# Autodesk Inventor assembly: Assembly
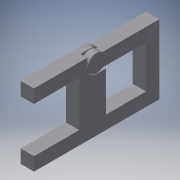
[picture p0: Inventor's stored thumbnail of the model, 180x180]
Saved by Autodesk Inventor 2019 (Build 230136000, 136)
## iProperties
Created: 2018-08-02
Part Number: Assembly
Document SubType Name: Assembly
Designer: zacha
Author: zacha
## Documents named in this file (3)
- F:\SkyDrive\Projects\Cable Guides\Home desk\Assembly.iam
- F:\SkyDrive\Projects\Cable Guides\Home desk\Main.ipt
- F:\SkyDrive\Projects\Cable Guides\Home desk\Latch.ipt
## Components (2 placed, 2 different names)
1. Main:1 — Flush:1
2. Latch:1 — Flush:1
## Relationships (1: Flush 1)
- Flush:1: Main:1 ↔ Latch:1
